# Autodesk Inventor assembly: Gehäusezusammenbau
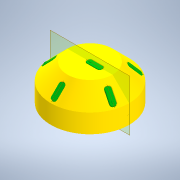
[picture p0: Inventor's stored thumbnail of the model, 180x180]
Saved by Autodesk Inventor 2020.2 (Build 242310000, 310)
## iProperties
Created: 2020-02-12
Part Number: Gehäusezusammenbau
Document SubType Name: Assembly
Designer: Max
Author: Max
## Documents named in this file (5)
- D:\Eigene Dateien\Dokumente\SynologyDrive\Uni\Studienarbeit\Eigene Inhalte\studienarbeitakustik\GehäuseCad\Gehäuse\Gehäusezusammenbau.iam
- D:\Eigene Dateien\Dokumente\SynologyDrive\Uni\Studienarbeit\Eigene Inhalte\studienarbeitakustik\GehäuseCad\Standardteile\Raspi 4\raspberry-pi-4B\Raspberry Pi 4 Model B.iam
- D:\Eigene Dateien\Dokumente\SynologyDrive\Uni\Studienarbeit\Eigene Inhalte\studienarbeitakustik\GehäuseCad\Gehäuse\GehaeuseteilA.ipt
- D:\Eigene Dateien\Dokumente\SynologyDrive\Uni\Studienarbeit\Eigene Inhalte\studienarbeitakustik\GehäuseCad\Standardteile\Mirofonboard\GehauseteilC.ipt
- D:\Eigene Dateien\Dokumente\SynologyDrive\Uni\Studienarbeit\Eigene Inhalte\studienarbeitakustik\GehäuseCad\Standardteile\Mirofonboard\Sensorboard.iam
## Components (11 placed, 4 different names)
1. Raspberry Pi 4 Model B:1 [sub-assembly] — Fluchtend:1
2. GehaeuseteilA:1 — Fluchtend:1, Fluchtend:2
3. GehauseteilC:1 — Fluchtend:2, Fluchtend:13, Fluchtend:16, Fluchtend:18, Fluchtend:19
4. Sensorboard:1 [sub-assembly] — Fluchtend:13, Passend:17, Fluchtend:16
5. Sensorboard:2 [sub-assembly] — Passend:18, Passend:19
6. Sensorboard:3 [sub-assembly]
7. Sensorboard:4 [sub-assembly]
8. Sensorboard:5 [sub-assembly]
9. Sensorboard:6 [sub-assembly] — Fluchtend:18
10. Sensorboard:7 [sub-assembly]
11. Sensorboard:8 [sub-assembly]
## Component patterns: (7 elements, first: Sensorboard:2)
## Relationships (29: Mate 16, Flush 10, Angle 3)
- Fluchtend:1 [Flush] (5 mm): Raspberry Pi 4 Model B:1 ↔ GehaeuseteilA:1
- Fluchtend:2 [Flush]: GehaeuseteilA:1 ↔ GehauseteilC:1
- Fluchtend:3 [Flush] (1.87 mm)
- Fluchtend:4 [Flush] (-1.563 mm)
- Fluchtend:6 [Flush] (31 mm)
- Passend:2 [Mate]
- Passend:3 [Mate]
- Passend:4 [Mate]
- Passend:5 [Mate]
- Winkel:2 [Angle] (0 deg)
- Passend:6 [Mate]
- Winkel:3 [Angle] (0 deg)
- Passend:7 [Mate]
- Fluchtend:15 [Flush] (-64.5 mm)
- Passend:8 [Mate]
- Passend:9 [Mate]
- Winkel:4 [Angle] (-45 deg)
- Passend:11 [Mate]
- Passend:12 [Mate]
- Passend:13 [Mate]
- Passend:14 [Mate]
- Passend:15 [Mate]
- Fluchtend:13 [Flush]: GehauseteilC:1 ↔ Sensorboard:1
- Passend:17 [Mate]: Sensorboard:1
- Passend:18 [Mate]: Sensorboard:2
- Passend:19 [Mate]: Sensorboard:2
- Fluchtend:16 [Flush]: GehauseteilC:1 ↔ Sensorboard:1
- Fluchtend:18 [Flush]: GehauseteilC:1 ↔ Sensorboard:6
- Fluchtend:19 [Flush]: GehauseteilC:1
